# Autodesk Inventor assembly: Chess Board
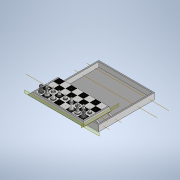
[picture p0: Inventor's stored thumbnail of the model, 180x180]
Saved by Autodesk Inventor 2022 (Build 260153000, 153)
## iProperties
Created: 2022-04-03
Part Number: Chess Board
Document SubType Name: Assembly
Designer: Nick
Author: Nick
## Documents named in this file (12)
- Y:\Projects\Chess_Board\Chess Board.iam
- Y:\Projects\Chess_Board\Top Base.ipt
- Y:\Projects\Chess_Board\Bottom Base.ipt
- Y:\Projects\Chess_Board\Board Pattern.iam
- Y:\Projects\Chess_Board\Angle Bracket.ipt
- Y:\Projects\Chess_Board\Linkage.ipt
- Y:\Projects\Chess_Board\Pieces\Pawn.ipt
- Y:\Projects\Chess_Board\Pieces\Rook.ipt
- Y:\Projects\Chess_Board\Pieces\Knight.ipt
- Y:\Projects\Chess_Board\M3 X 6mm BHCS.ipt
- Y:\Projects\Chess_Board\M3 Acorn Nut.ipt
- Y:\Projects\Chess_Board\Bishop.ipt
## Components (37 placed, 11 different names)
1. Top Base:2 — Mate:11, Mate:12, Mate:13, Mate:14, Mate:59, Mate:60, Mate:61, Mate:62, Flush:7
2. Bottom Base:1 — Mate:11, Mate:27, Mate:28, Mate:31, Mate:32, Angle:5, Mate:67, Mate:69
3. Board Pattern:2 [sub-assembly] — Mate:12, Mate:13, Mate:14, Mate:35, Mate:36, Mate:37, Mate:38, Mate:39, Mate:40, Mate:41, Mate:42, Mate:43, Mate:44, Mate:45, Mate:46, Mate:47, Mate:48, Mate:49, Mate:50, Mate:51, Mate:52, Mate:53, Mate:54, Mate:55, Mate:56, Mate:57, Mate:58, Mate:70, Mate:71, Mate:72, Mate:73
4. Angle Bracket:5 — Mate:60, Insert:18
5. Angle Bracket:6 — Mate:59, Insert:17
6. Linkage:6 — Flush:6, Mate:32, Angle:7, Insert:13, Insert:17, Insert:22
7. Linkage:7 — Flush:6, Mate:31, Insert:14, Insert:18, Insert:21
8. Angle Bracket:7 — Mate:61, Insert:16, Flush:7
9. Angle Bracket:8 — Mate:62, Insert:15
10. Linkage:8 — Flush:5, Mate:27, Insert:11, Insert:15, Insert:25
11. Linkage:9 — Flush:5, Mate:28, Angle:7, Insert:12, Insert:16, Insert:26
12. Pawn:1 — Mate:35, Mate:36
13. Pawn:2 — Mate:40, Mate:47
14. Pawn:3 — Mate:41, Mate:50
15. Pawn:4 — Mate:37, Mate:46
16. Pawn:5 — Mate:39, Mate:45
17. Pawn:6 — Mate:38, Mate:44
18. Pawn:7 — Mate:43, Mate:48
19. Pawn:8 — Mate:42, Mate:49
20. Rook:1 — Mate:52, Mate:53
21. Rook:2 — Mate:51, Mate:54
22. Knight:1 — Mate:56, Mate:58, Angle:5, Angle:6
23. Knight:2 — Mate:55, Mate:57, Angle:6
24. Angle Bracket:9 — Insert:12, Insert:24, Mate:69
25. Angle Bracket:10 — Insert:11, Insert:23
26. Angle Bracket:11 — Insert:14, Insert:20
27. Angle Bracket:12 — Insert:13, Insert:19, Mate:67
28. M3 X 6mm BHCS:1 — Insert:20
29. M3 X 6mm BHCS:2 — Insert:19
30. M3 Acorn Nut:1 — Insert:21
31. M3 Acorn Nut:2 — Insert:22
32. M3 X 6mm BHCS:3 — Insert:24
33. M3 X 6mm BHCS:4 — Insert:23
34. M3 Acorn Nut:3 — Insert:25
35. M3 Acorn Nut:4 — Insert:26
36. Bishop:1 — Mate:70, Mate:73
37. Bishop:2 — Mate:71, Mate:72
## Relationships (66: Mate 42, Insert 16, Angle 5, Flush 3)
- Mate:11: Top Base:2 ↔ Bottom Base:1
- Mate:12: Top Base:2 ↔ Board Pattern:2
- Mate:13: Top Base:2 ↔ Board Pattern:2
- Mate:14: Top Base:2 ↔ Board Pattern:2
- [Angle] (180 deg): Linkage:6 ↔ Linkage:7
- [Angle] (180 deg): Linkage:8 ↔ Linkage:9
- Flush:5: Linkage:8 ↔ Linkage:9
- Flush:6: Linkage:6 ↔ Linkage:7
- Mate:27: Bottom Base:1 ↔ Linkage:8
- Mate:28: Bottom Base:1 ↔ Linkage:9
- Mate:31: Bottom Base:1 ↔ Linkage:7
- Mate:32: Bottom Base:1 ↔ Linkage:6
- Mate:35: Board Pattern:2 ↔ Pawn:1
- Mate:36: Board Pattern:2 ↔ Pawn:1
- Mate:37: Board Pattern:2 ↔ Pawn:4
- Mate:38: Board Pattern:2 ↔ Pawn:6
- Mate:39: Board Pattern:2 ↔ Pawn:5
- Mate:40: Board Pattern:2 ↔ Pawn:2
- Mate:41: Board Pattern:2 ↔ Pawn:3
- Mate:42: Board Pattern:2 ↔ Pawn:8
- Mate:43: Board Pattern:2 ↔ Pawn:7
- Mate:44: Board Pattern:2 ↔ Pawn:6
- Mate:45: Board Pattern:2 ↔ Pawn:5
- Mate:46: Board Pattern:2 ↔ Pawn:4
- Mate:47: Board Pattern:2 ↔ Pawn:2
- Mate:48: Board Pattern:2 ↔ Pawn:7
- Mate:49: Board Pattern:2 ↔ Pawn:8
- Mate:50: Board Pattern:2 ↔ Pawn:3
- Mate:51: Board Pattern:2 ↔ Rook:2
- Mate:52: Board Pattern:2 ↔ Rook:1
- Mate:53: Board Pattern:2 ↔ Rook:1
- Mate:54: Board Pattern:2 ↔ Rook:2
- Mate:55: Board Pattern:2 ↔ Knight:2
- Mate:56: Board Pattern:2 ↔ Knight:1
- Mate:57: Board Pattern:2 ↔ Knight:2
- Mate:58: Board Pattern:2 ↔ Knight:1
- Angle:5 (180 deg): Bottom Base:1 ↔ Knight:1
- Angle:6 (0 deg): Knight:1 ↔ Knight:2
- Mate:59: Top Base:2 ↔ Angle Bracket:6
- Mate:60: Top Base:2 ↔ Angle Bracket:5
- Mate:61: Top Base:2 ↔ Angle Bracket:7
- Mate:62: Top Base:2 ↔ Angle Bracket:8
- Angle:7 (0 deg): Linkage:6 ↔ Linkage:9
- Insert:11 (1 mm): Linkage:8 ↔ Angle Bracket:10
- Insert:12 (1 mm): Linkage:9 ↔ Angle Bracket:9
- Insert:13 (1 mm): Linkage:6 ↔ Angle Bracket:12
- Insert:14 (1 mm): Linkage:7 ↔ Angle Bracket:11
- Insert:15 (1 mm): Angle Bracket:8 ↔ Linkage:8
- Insert:16 (1 mm): Angle Bracket:7 ↔ Linkage:9
- Insert:17 (1 mm): Angle Bracket:6 ↔ Linkage:6
- Insert:18 (1 mm): Angle Bracket:5 ↔ Linkage:7
- Insert:19: Angle Bracket:12 ↔ M3 X 6mm BHCS:2
- Insert:20: Angle Bracket:11 ↔ M3 X 6mm BHCS:1
- Insert:21: Linkage:7 ↔ M3 Acorn Nut:1
- Insert:22: Linkage:6 ↔ M3 Acorn Nut:2
- Mate:67 (2 mm): Bottom Base:1 ↔ Angle Bracket:12
- Insert:23: Angle Bracket:10 ↔ M3 X 6mm BHCS:4
- Insert:24: Angle Bracket:9 ↔ M3 X 6mm BHCS:3
- Insert:25: Linkage:8 ↔ M3 Acorn Nut:3
- Insert:26: Linkage:9 ↔ M3 Acorn Nut:4
- Mate:69 (2 mm): Bottom Base:1 ↔ Angle Bracket:9
- Flush:7 (3.511 mm): Top Base:2 ↔ Angle Bracket:7
- Mate:70: Board Pattern:2 ↔ Bishop:1
- Mate:71: Board Pattern:2 ↔ Bishop:2
- Mate:72: Board Pattern:2 ↔ Bishop:2
- Mate:73: Board Pattern:2 ↔ Bishop:1
## Named parameters: d95_d91_d77 = 180 deg, d99_d91_d77 = 180 deg
